# Autodesk Inventor assembly: Assembly1
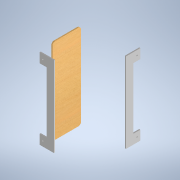
[picture p0: Inventor's stored thumbnail of the model, 180x180]
Saved by Autodesk Inventor 2022.2 (Build 262287000, 287)
## iProperties
Created: 2022-03-14
Part Number: Assembly1
Document SubType Name: Assembly
Designer: PRASHANTH
Author: PRASHANTH
## Documents named in this file (3)
- E:\BME\Autodesk Sample\Engg Exploration\Subsystem1-Conveyor Belt\Assembly1.iam
- E:\BME\Autodesk Sample\Engg Exploration\Subsystem1-Conveyor Belt\Conveyor Base.ipt
- E:\BME\Autodesk Sample\Engg Exploration\Subsystem1-Conveyor Belt\Conveyor Support.ipt
## Components (3 placed, 2 different names)
1. Conveyor Base:1 — Mate:1
2. Conveyor Support:1 — Mate:1
3. Conveyor Support:2
## Relationships (1: Mate 1)
- Mate:1: Conveyor Base:1 ↔ Conveyor Support:1
